# Autodesk Inventor assembly: FourPartTelescopeV2
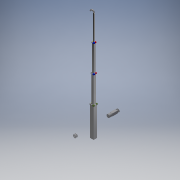
[picture p0: Inventor's stored thumbnail of the model, 180x180]
Saved by Autodesk Inventor 2018.3 (Build 223284000, 284)
## iProperties
Created: 2020-01-18
Part Number: FourPartTelescopeV2
Document SubType Name: Assembly
Designer: Cooper
Mass: 1531.34 g
Surface Area: 7090.2 cm^2
Volume: 590.258 cm^3
Density: 2.59435 g/cm^3
Author: Cooper
## Documents named in this file (18)
- C:\Users\22perngrac\Documents\GrabCAD\Infinite Recharge 2020\Build season\CLB_001_FourPartTelescope.iam
- C:\Users\22perngrac\Documents\GrabCAD\Infinite Recharge 2020\Build season\CLB_002_TelescopeInnerBarS1.ipt
- C:\Users\22perngrac\Documents\GrabCAD\Infinite Recharge 2020\Build season\CLB_003_TelescopeMiddleBarS2.ipt
- C:\Users\22perngrac\Documents\GrabCAD\Infinite Recharge 2020\Build season\CLB_004_TelescopeOuterBars3.ipt
- C:\Users\22perngrac\Documents\GrabCAD\Infinite Recharge 2020\Build season\CLB_005_TelescopeHook.ipt
- C:\Users\22perngrac\Documents\GrabCAD\Infinite Recharge 2020\Build season\CLB_006_TelescopeOuterBarS4.ipt
- C:\Users\22perngrac\Documents\GrabCAD\Infinite Recharge 2020\Build season\CLB_007_TelescopePlug1.75.ipt
- C:\Users\22perngrac\Documents\GrabCAD\Infinite Recharge 2020\Build season\CLB_008_TelescopePlug.ipt
- C:\Users\22perngrac\Documents\GrabCAD\Infinite Recharge 2020\Build season\CLB_017_8TelescopeGroot.ipt
- C:\Users\22perngrac\Documents\GrabCAD\Infinite Recharge 2020\Build season\CLB_018_16GrootTelescopeLeft.ipt
- C:\Users\22perngrac\Documents\GrabCAD\Infinite Recharge 2020\Build season\CLB_019_16GrootTelescopeRight.ipt
- C:\Users\22perngrac\Documents\GrabCAD\Infinite Recharge 2020\Build season\CLB_020_TelescopeS1Plug.ipt
- C:\Users\22perngrac\Documents\GrabCAD\Infinite Recharge 2020\Build season\CLB_021_ScissorLiftMotorApproximation.ipt
- C:\Users\22perngrac\Documents\GrabCAD\Infinite Recharge 2020\Build season\CLB_022_PulleySurface.ipt
- C:\Users\22perngrac\Documents\GrabCAD\Infinite Recharge 2020\Build season\CLB_023_RollerAssembly(Bearing)S2.iam
- C:\Users\22perngrac\Documents\GrabCAD\Infinite Recharge 2020\Build season\CLB_024_RollerAssembly(Bearing)S3.iam
- C:\Users\22perngrac\Documents\GrabCAD\Infinite Recharge 2020\Build season\CLB_025_RollerAssembly(Bearing)S4.iam
- C:\Users\22perngrac\Documents\GrabCAD\Infinite Recharge 2020\Brainstorming\Climber\CLB_Winch_Rear.ipt
## Components (21 placed, 17 different names)
1. CLB_002_TelescopeInnerBarS1:1 — Mate:4, Mate:5, Mate:6, Mate:20, Mate:27, Mate:56, Mate:57, Mate:60, Mate:61, Mate:68
2. CLB_003_TelescopeMiddleBarS2:1 — Mate:11, Mate:16, Flush:16, Mate:17, Flush:17, Mate:19, Mate:20, Mate:24, Mate:25, Mate:41, Mate:44, Mate:46, Mate:48, Mate:49, Mate:50, Mate:60
3. CLB_004_TelescopeOuterBars3:1 — Mate:10, Mate:14, Flush:15, Mate:15, Flush:17, Mate:18, Mate:19, Mate:22, Mate:23, Mate:35, Mate:38, Mate:51, Mate:52, Mate:53, Mate:54
4. CLB_005_TelescopeHook:1 — Mate:5, Mate:6, Mate:27
5. CLB_006_TelescopeOuterBarS4:1 — Mate:8, Mate:9, Flush:9, Mate:12, Flush:14, Mate:13, Mate:18, Flush:19, Mate:28, Mate:29, Mate:30, Mate:31, Mate:32, Mate:33, Mate:63
6. CLB_007_TelescopePlug1.75:1 — Mate:10, Mate:22, Mate:23, Mate:26, Flush:19, Mate:34, Mate:63, Mate:66, Mate:70
7. CLB_008_TelescopePlug:1 — Mate:11, Mate:24, Mate:25, Mate:4, Mate:26, Mate:55, Mate:65, Mate:67, Mate:69
8. CLB_023_RollerAssembly(Bearing)S2:1 [sub-assembly] — Mate:16, Flush:16, Mate:17
9. CLB_024_RollerAssembly(Bearing)S3:1 [sub-assembly] — Mate:14, Flush:15, Mate:15
10. CLB_025_RollerAssembly(Bearing)S4:1 [sub-assembly] — Mate:12, Flush:14, Mate:13
11. CLB_017_8TelescopeGroot:1 — Mate:31, Mate:32, Mate:33
12. CLB_017_8TelescopeGroot:2 — Mate:28, Mate:29, Mate:30, Mate:34, Mate:64
13. CLB_018_16GrootTelescopeLeft:1 — Mate:38, Mate:51, Mate:52, Mate:64
14. CLB_019_16GrootTelescopeRight:1 — Mate:35, Mate:53, Mate:54, Mate:55
15. CLB_018_16GrootTelescopeLeft:2 — Mate:41, Mate:46, Mate:50, Mate:62
16. CLB_019_16GrootTelescopeRight:2 — Mate:44, Mate:48, Mate:49
17. CLB_020_TelescopeS1Plug:1 — Mate:56, Mate:57, Mate:61, Mate:62, Mate:65, Mate:68
18. CLB_021_ScissorLiftMotorApproximation:1
19. CLB_022_PulleySurface:1 — Mate:66, Mate:70
20. CLB_022_PulleySurface:2 — Mate:67, Mate:69
21. CLB_Winch_Rear:1
## Relationships (61: Mate 55, Flush 6)
- Mate:4: CLB_002_TelescopeInnerBarS1:1 ↔ CLB_008_TelescopePlug:1
- Mate:5: CLB_002_TelescopeInnerBarS1:1 ↔ CLB_005_TelescopeHook:1
- Mate:6: CLB_002_TelescopeInnerBarS1:1 ↔ CLB_005_TelescopeHook:1
- Mate:8: CLB_006_TelescopeOuterBarS4:1
- Mate:9: CLB_006_TelescopeOuterBarS4:1
- Flush:9: CLB_006_TelescopeOuterBarS4:1
- Mate:10: CLB_004_TelescopeOuterBars3:1 ↔ CLB_007_TelescopePlug1.75:1
- Mate:11: CLB_003_TelescopeMiddleBarS2:1 ↔ CLB_008_TelescopePlug:1
- Mate:12: CLB_006_TelescopeOuterBarS4:1 ↔ CLB_025_RollerAssembly(Bearing)S4:1
- Flush:14: CLB_006_TelescopeOuterBarS4:1 ↔ CLB_025_RollerAssembly(Bearing)S4:1
- Mate:13 (3.175 mm): CLB_006_TelescopeOuterBarS4:1 ↔ CLB_025_RollerAssembly(Bearing)S4:1
- Mate:14: CLB_004_TelescopeOuterBars3:1 ↔ CLB_024_RollerAssembly(Bearing)S3:1
- Flush:15: CLB_004_TelescopeOuterBars3:1 ↔ CLB_024_RollerAssembly(Bearing)S3:1
- Mate:15 (3.175 mm): CLB_004_TelescopeOuterBars3:1 ↔ CLB_024_RollerAssembly(Bearing)S3:1
- Mate:16: CLB_003_TelescopeMiddleBarS2:1 ↔ CLB_023_RollerAssembly(Bearing)S2:1
- Flush:16: CLB_003_TelescopeMiddleBarS2:1 ↔ CLB_023_RollerAssembly(Bearing)S2:1
- Mate:17 (3.175 mm): CLB_003_TelescopeMiddleBarS2:1 ↔ CLB_023_RollerAssembly(Bearing)S2:1
- Flush:17 (3.175 mm): CLB_003_TelescopeMiddleBarS2:1 ↔ CLB_004_TelescopeOuterBars3:1
- Mate:18 (6.35 mm): CLB_004_TelescopeOuterBars3:1 ↔ CLB_006_TelescopeOuterBarS4:1
- Mate:19 (4.7625 mm): CLB_003_TelescopeMiddleBarS2:1 ↔ CLB_004_TelescopeOuterBars3:1
- Mate:20 (4.7625 mm): CLB_002_TelescopeInnerBarS1:1 ↔ CLB_003_TelescopeMiddleBarS2:1
- Mate:22: CLB_004_TelescopeOuterBars3:1 ↔ CLB_007_TelescopePlug1.75:1
- Mate:23: CLB_004_TelescopeOuterBars3:1 ↔ CLB_007_TelescopePlug1.75:1
- Mate:24: CLB_003_TelescopeMiddleBarS2:1 ↔ CLB_008_TelescopePlug:1
- Mate:25: CLB_003_TelescopeMiddleBarS2:1 ↔ CLB_008_TelescopePlug:1
- Mate:26: CLB_007_TelescopePlug1.75:1 ↔ CLB_008_TelescopePlug:1
- Flush:19: CLB_006_TelescopeOuterBarS4:1 ↔ CLB_007_TelescopePlug1.75:1
- Mate:27: CLB_002_TelescopeInnerBarS1:1 ↔ CLB_005_TelescopeHook:1
- Mate:28: CLB_006_TelescopeOuterBarS4:1 ↔ CLB_017_8TelescopeGroot:2
- Mate:29: CLB_006_TelescopeOuterBarS4:1 ↔ CLB_017_8TelescopeGroot:2
- Mate:30: CLB_006_TelescopeOuterBarS4:1 ↔ CLB_017_8TelescopeGroot:2
- Mate:31: CLB_006_TelescopeOuterBarS4:1 ↔ CLB_017_8TelescopeGroot:1
- Mate:32: CLB_006_TelescopeOuterBarS4:1 ↔ CLB_017_8TelescopeGroot:1
- Mate:33: CLB_006_TelescopeOuterBarS4:1 ↔ CLB_017_8TelescopeGroot:1
- Mate:34: CLB_007_TelescopePlug1.75:1 ↔ CLB_017_8TelescopeGroot:2
- Mate:35: CLB_004_TelescopeOuterBars3:1 ↔ CLB_019_16GrootTelescopeRight:1
- Mate:38: CLB_004_TelescopeOuterBars3:1 ↔ CLB_018_16GrootTelescopeLeft:1
- Mate:41: CLB_003_TelescopeMiddleBarS2:1 ↔ CLB_018_16GrootTelescopeLeft:2
- Mate:44: CLB_003_TelescopeMiddleBarS2:1 ↔ CLB_019_16GrootTelescopeRight:2
- Mate:46: CLB_003_TelescopeMiddleBarS2:1 ↔ CLB_018_16GrootTelescopeLeft:2
- Mate:48: CLB_003_TelescopeMiddleBarS2:1 ↔ CLB_019_16GrootTelescopeRight:2
- Mate:49: CLB_003_TelescopeMiddleBarS2:1 ↔ CLB_019_16GrootTelescopeRight:2
- Mate:50: CLB_003_TelescopeMiddleBarS2:1 ↔ CLB_018_16GrootTelescopeLeft:2
- Mate:51: CLB_004_TelescopeOuterBars3:1 ↔ CLB_018_16GrootTelescopeLeft:1
- Mate:52: CLB_004_TelescopeOuterBars3:1 ↔ CLB_018_16GrootTelescopeLeft:1
- Mate:53: CLB_004_TelescopeOuterBars3:1 ↔ CLB_019_16GrootTelescopeRight:1
- Mate:54: CLB_004_TelescopeOuterBars3:1 ↔ CLB_019_16GrootTelescopeRight:1
- Mate:55: CLB_008_TelescopePlug:1 ↔ CLB_019_16GrootTelescopeRight:1
- Mate:56: CLB_002_TelescopeInnerBarS1:1 ↔ CLB_020_TelescopeS1Plug:1
- Mate:57: CLB_002_TelescopeInnerBarS1:1 ↔ CLB_020_TelescopeS1Plug:1
- Mate:60 (6.35 mm): CLB_002_TelescopeInnerBarS1:1 ↔ CLB_003_TelescopeMiddleBarS2:1
- Mate:61: CLB_002_TelescopeInnerBarS1:1 ↔ CLB_020_TelescopeS1Plug:1
- Mate:62: CLB_018_16GrootTelescopeLeft:2 ↔ CLB_020_TelescopeS1Plug:1
- Mate:63 (9.525 mm): CLB_006_TelescopeOuterBarS4:1 ↔ CLB_007_TelescopePlug1.75:1
- Mate:64: CLB_017_8TelescopeGroot:2 ↔ CLB_018_16GrootTelescopeLeft:1
- Mate:65: CLB_008_TelescopePlug:1 ↔ CLB_020_TelescopeS1Plug:1
- Mate:66: CLB_007_TelescopePlug1.75:1 ↔ CLB_022_PulleySurface:1
- Mate:67: CLB_008_TelescopePlug:1 ↔ CLB_022_PulleySurface:2
- Mate:68: CLB_002_TelescopeInnerBarS1:1 ↔ CLB_020_TelescopeS1Plug:1
- Mate:69: CLB_008_TelescopePlug:1 ↔ CLB_022_PulleySurface:2
- Mate:70: CLB_007_TelescopePlug1.75:1 ↔ CLB_022_PulleySurface:1
